# Autodesk Inventor assembly: OUTK_000_Assembly
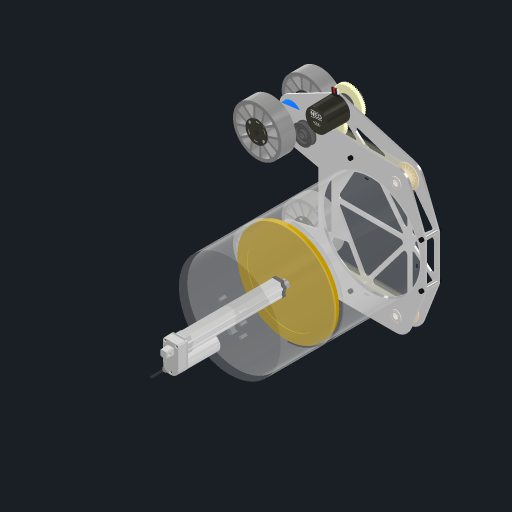
[picture p0: Inventor's stored thumbnail of the model, 512x512]
Saved by Autodesk Inventor 2024.2 (Build 282272000, 272)
## iProperties
Created: 2024-11-24
Part Number: OUTK_000_Assembly
Document SubType Name: Assembly
Designer: Bryan
Mass: 9682.5 g
Surface Area: 20203.5 cm^2
Volume: 5331.75 cm^3
Density: 1.81601 g/cm^3
Author: Bryan
## Documents named in this file (23)
- C:\Users\bobsb\OneDrive\Documents\GitHub\1622-2024-Casino-Clash-CAD-A-Thon\Outtake\OUTK_000_Assembly.iam
- C:\Users\bobsb\OneDrive\Documents\GitHub\1622-2024-Casino-Clash-CAD-A-Thon\Outtake\OUTK_002_ShotPlateNoReceptacle.ipt
- C:\Users\bobsb\OneDrive\Documents\GitHub\1622-2024-Casino-Clash-CAD-A-Thon\Outtake\OUTK_002_ShotPlateReceptacle.ipt
- C:\Users\bobsb\OneDrive\Documents\GitHub\1622-2024-Casino-Clash-CAD-A-Thon\Outtake\OUTK_001_ChipBucket.ipt
- C:\Users\bobsb\OneDrive\Documents\GitHub\1622-2024-Casino-Clash-CAD-A-Thon\COTS Library\Motion\Linear Actuators\PA-01\COTS_PA-01.iam
- C:\Users\bobsb\OneDrive\Documents\GitHub\1622-2024-Casino-Clash-CAD-A-Thon\COTS Library\Motion\Linear Actuators\PA-01\Shaft.ipt
- C:\Users\bobsb\OneDrive\Documents\GitHub\1622-2024-Casino-Clash-CAD-A-Thon\COTS Library\Motion\Bearings\COTS_WCP-0783_1.125ODHexBearing.ipt
- C:\Users\bobsb\OneDrive\Documents\GitHub\1622-2024-Casino-Clash-CAD-A-Thon\COTS Library\Motion\Wheels\Compliant Wheels\5in compliant wheels\COTS_5 Straight Flex Wheel (.ipt
- C:\Users\bobsb\OneDrive\Documents\GitHub\1622-2024-Casino-Clash-CAD-A-Thon\COTS Library\Adapters\COTS_1_2” Hex Bore Aluminum VersaHub (217-2592)(1).ipt
- C:\Users\bobsb\OneDrive\Documents\GitHub\1622-2024-Casino-Clash-CAD-A-Thon\COTS Library\Motion\Wheels\Compliant Wheels\2in compliant wheels\0.500in hex bore\COTS_am-3462_2indiameter_0.500inhexbore_durometer50A_CompliantWheel.ipt
- C:\Users\bobsb\OneDrive\Documents\GitHub\1622-2024-Casino-Clash-CAD-A-Thon\Game Objects\Chip, Simplified.ipt
- C:\Users\bobsb\OneDrive\Documents\GitHub\1622-2024-Casino-Clash-CAD-A-Thon\Outtake\OUTK_010_Grippy.ipt
- C:\Users\bobsb\OneDrive\Documents\GitHub\1622-2024-Casino-Clash-CAD-A-Thon\Outtake\OUTK_011_Tubing.ipt
- C:\Users\bobsb\OneDrive\Documents\GitHub\1622-2024-Casino-Clash-CAD-A-Thon\COTS Library\Fasteners\Bolts\Set Screws\10-32\COTS_91375A446_Alloy Steel Cup-Point Set Screw.ipt
- C:\Users\bobsb\OneDrive\Documents\GitHub\1622-2024-Casino-Clash-CAD-A-Thon\COTS Library\Motion\Pulleys\HTD5M\10mm Wide\COTS_30T_WCP-0565.ipt
- C:\Users\bobsb\OneDrive\Documents\GitHub\1622-2024-Casino-Clash-CAD-A-Thon\COTS Library\Motors\COTS_REV-21-1650-V1.1_Neo1.1.ipt
- C:\Users\bobsb\OneDrive\Documents\GitHub\1622-2024-Casino-Clash-CAD-A-Thon\COTS Library\Fasteners\Bolts\Button-Head\10-32\COTS_91255A265_Button Head Hex Drive Screw.ipt
- C:\Users\bobsb\OneDrive\Documents\GitHub\1622-2024-Casino-Clash-CAD-A-Thon\COTS Library\Adapters\COTS_REV-21-1879_8mmKeyTo0.5Hex.ipt
- C:\Users\bobsb\OneDrive\Documents\GitHub\1622-2024-Casino-Clash-CAD-A-Thon\COTS Library\Motion\Pulleys\HTD5M\10mm Wide\COTS_24T_WCP-0564.ipt
- C:\Users\bobsb\OneDrive\Documents\GitHub\1622-2024-Casino-Clash-CAD-A-Thon\COTS Library\Motion\Gears\20DP gears\Aluminum\0.5in hex\COTS_60T_WCP-0720(1).ipt
- C:\Users\bobsb\OneDrive\Documents\GitHub\1622-2024-Casino-Clash-CAD-A-Thon\Outtake\OUTK_012_Spacer1.ipt
- C:\Users\bobsb\OneDrive\Documents\GitHub\1622-2024-Casino-Clash-CAD-A-Thon\Outtake\OUTK_013_Standoff1.ipt
- C:\Users\bobsb\OneDrive\Documents\GitHub\1622-2024-Casino-Clash-CAD-A-Thon\COTS Library\Fasteners\Bolts\Socket-Head\0.25-20\COTS_91251A537_Black-Oxide Alloy Steel Socket Head Screw_.25-20_.5in.ipt
## Components (116 placed, 22 different names)
1. OUTK_002_ShotPlateNoReceptacle:1 — Mate:4, Mate:5, Mate:41, Mate:47, Mate:50, Mate:52, Mate:55, Mate:56, Mate:57, Mate:65, Mate:66, Mate:67, Mate:68, Mate:69, Mate:70, Mate:149, Mate:150, Mate:151, Mate:152, Mate:153, Mate:169, Mate:170, Mate:171, Mate:172, Mate:173, Mate:174, Mate:175, Mate:176, Mate:177, Mate:178, Mate:181, Mate:182, Mate:187, Mate:188, Mate:189, Mate:192
2. OUTK_002_ShotPlateReceptacle:1 — Mate:3, Mate:4, Mate:5, Mate:41, Mate:42, Mate:48, Mate:49, Mate:51, Mate:53, Mate:54, Mate:58, Mate:59, Mate:60, Mate:61, Mate:62, Mate:63, Mate:64, Mate:141, Mate:179, Mate:180, Mate:183, Mate:184, Mate:185, Mate:186, Mate:190, Mate:191
3. OUTK_001_ChipBucket:1 — Mate:3, Mate:42, Mate:43, Mate:44, Mate:114, Flush:1, Mate:161, Mate:162
4. COTS_PA-01:1 [sub-assembly] — Mate:43, Mate:44, Mate:46, Flush:1
5. Shaft:1 — Mate:46, Mate:115
6. COTS_WCP-0783_1.125ODHexBearing:1 — Mate:47, Mate:65, Mate:72, Mate:107, Mate:166, Mate:168
7. COTS_WCP-0783_1.125ODHexBearing:2 — Mate:48, Mate:62, Mate:74, Mate:106, Mate:108, Mate:145
8. COTS_WCP-0783_1.125ODHexBearing:3 — Mate:49, Mate:64, Mate:120, Mate:143, Mate:146
9. COTS_WCP-0783_1.125ODHexBearing:4 — Mate:50, Mate:66, Mate:124, Mate:156, Mate:157
10. COTS_WCP-0783_1.125ODHexBearing:5 — Mate:51, Mate:63, Mate:117
11. COTS_WCP-0783_1.125ODHexBearing:6 — Mate:52, Mate:67, Mate:123
12. COTS_WCP-0783_1.125ODHexBearing:7 — Mate:55, Mate:69, Mate:122, Mate:160
13. COTS_WCP-0783_1.125ODHexBearing:8 — Mate:56, Mate:68, Mate:71, Mate:110, Mate:111, Mate:163, Mate:165
14. COTS_WCP-0783_1.125ODHexBearing:9 — Mate:53, Mate:61, Mate:119, Mate:142, Mate:144
15. COTS_WCP-0783_1.125ODHexBearing:10 — Mate:54, Mate:60, Mate:73, Mate:112, Mate:139, Mate:140
16. COTS_WCP-0783_1.125ODHexBearing:11 — Mate:57, Mate:70, Mate:121
17. COTS_WCP-0783_1.125ODHexBearing:12 — Mate:58, Mate:59, Mate:118
18. COTS_5 Straight Flex Wheel (:1 — Mate:71, Mate:75, Mate:80, Mate:85, Mate:88, Mate:89, Mate:90
19. COTS_5 Straight Flex Wheel (:2 — Mate:72, Mate:76, Mate:81, Mate:86, Mate:87, Mate:94, Mate:95, Mate:96
20. COTS_5 Straight Flex Wheel (:3 — Mate:73, Mate:78, Mate:79, Mate:84, Mate:91, Mate:92, Mate:93
21. COTS_5 Straight Flex Wheel (:4 — Mate:74, Mate:77, Mate:82, Mate:83, Mate:97, Mate:98, Mate:99
22. COTS_1_2” Hex Bore Aluminum VersaHub (217-2592)(1):1 — Mate:77, Mate:82, Mate:83, Mate:135, Flush:8
23. COTS_1_2” Hex Bore Aluminum VersaHub (217-2592)(1):2 — Mate:76, Mate:81, Mate:86, Mate:87, Mate:130, Flush:3
24. COTS_1_2” Hex Bore Aluminum VersaHub (217-2592)(1):3 — Mate:78, Mate:79, Mate:84, Mate:134, Flush:7
25. COTS_1_2” Hex Bore Aluminum VersaHub (217-2592)(1):4 — Mate:75, Mate:80, Mate:85, Mate:131, Flush:4
26. COTS_1_2” Hex Bore Aluminum VersaHub (217-2592)(1):5 — Mate:88, Mate:89, Mate:90, Mate:132, Flush:5, Mate:164
27. COTS_1_2” Hex Bore Aluminum VersaHub (217-2592)(1):6 — Mate:91, Mate:92, Mate:93, Mate:133, Flush:6, Mate:147
28. COTS_1_2” Hex Bore Aluminum VersaHub (217-2592)(1):7 — Mate:94, Mate:95, Mate:96, Mate:129, Flush:2, Mate:167
29. COTS_1_2” Hex Bore Aluminum VersaHub (217-2592)(1):8 — Mate:97, Mate:98, Mate:99, Mate:136, Flush:9, Mate:148
30. COTS_am-3462_2indiameter_0.500inhexbore_durometer50A_CompliantWheel:1 — Mate:106, Mate:107, Mate:109
31. COTS_am-3462_2indiameter_0.500inhexbore_durometer50A_CompliantWheel:2 — Mate:108, Mate:109
32. COTS_am-3462_2indiameter_0.500inhexbore_durometer50A_CompliantWheel:3 — Mate:110, Mate:111, Mate:113
33. COTS_am-3462_2indiameter_0.500inhexbore_durometer50A_CompliantWheel:4 — Mate:112, Mate:113
34. Chip, Simplified:1 — Mate:114, Mate:115
35. OUTK_010_Grippy:1 — Mate:120, Mate:124, Mate:128
36. OUTK_010_Grippy:2 — Mate:119, Mate:122, Mate:126
37. OUTK_010_Grippy:3 — Mate:118, Mate:121, Mate:125, Tangent:4
38. OUTK_010_Grippy:4 — Mate:117, Mate:123, Mate:127, Tangent:5
39. OUTK_011_Tubing:1 — Mate:125, Mate:126, Tangent:4
40. OUTK_011_Tubing:2 — Mate:127, Mate:128, Tangent:5
41. COTS_30T_WCP-0565:1 — Mate:139, Mate:140, Mate:147
42. COTS_30T_WCP-0565:2 — Mate:141, Mate:145, Mate:148
43. COTS_30T_WCP-0565:3 — Mate:143, Mate:146
44. COTS_30T_WCP-0565:4 — Mate:142, Mate:144
45. COTS_REV-21-1650-V1.1_Neo1.1:1 — Mate:149, Mate:150, Mate:151, Mate:154, Mate:155, Mate:158
46. COTS_REV-21-1879_8mmKeyTo0.5Hex:1 — Mate:154, Flush:11
47. COTS_24T_WCP-0564:1 — Mate:155, Flush:10, Mate:159
48. COTS_24T_WCP-0564:2 — Mate:156, Mate:157, Flush:10
49. COTS_60T_WCP-0720(1):1 — Mate:158, Mate:159, Flush:11, Flush:12
50. COTS_60T_WCP-0720(1):2 — Mate:160, Flush:12
51. OUTK_012_Spacer1:1 — Mate:166, Mate:167, Mate:168
52. OUTK_012_Spacer1:2 — Mate:163, Mate:164, Mate:165
53. OUTK_013_Standoff1:1 — Mate:172, Mate:173
54. OUTK_013_Standoff1:2 — Mate:171, Mate:174
55. OUTK_013_Standoff1:3 — Mate:170, Mate:175
56. OUTK_013_Standoff1:4 — Mate:169, Mate:176
57. COTS_91251A537_Black-Oxide Alloy Steel Socket Head Screw_.25-20_.5in:1 — Mate:177, Mate:178
58. COTS_91251A537_Black-Oxide Alloy Steel Socket Head Screw_.25-20_.5in:2 — Mate:179, Mate:180
59. COTS_91251A537_Black-Oxide Alloy Steel Socket Head Screw_.25-20_.5in:3 — Mate:181, Mate:182
60. COTS_91251A537_Black-Oxide Alloy Steel Socket Head Screw_.25-20_.5in:4 — Mate:183, Mate:184
61. COTS_91251A537_Black-Oxide Alloy Steel Socket Head Screw_.25-20_.5in:5 — Mate:187, Mate:188
62. COTS_91251A537_Black-Oxide Alloy Steel Socket Head Screw_.25-20_.5in:6 — Mate:185, Mate:186
63. COTS_91251A537_Black-Oxide Alloy Steel Socket Head Screw_.25-20_.5in:7 — Mate:189, Mate:192
64. COTS_91251A537_Black-Oxide Alloy Steel Socket Head Screw_.25-20_.5in:8 — Mate:190, Mate:191
65. COTS_91375A446_Alloy Steel Cup-Point Set Screw:13 — Mate:129, Flush:2
66. COTS_91375A446_Alloy Steel Cup-Point Set Screw:14
67. COTS_91375A446_Alloy Steel Cup-Point Set Screw:15
68. COTS_91375A446_Alloy Steel Cup-Point Set Screw:16
69. COTS_91375A446_Alloy Steel Cup-Point Set Screw:17
70. COTS_91375A446_Alloy Steel Cup-Point Set Screw:18
71. COTS_91375A446_Alloy Steel Cup-Point Set Screw:1 — Mate:130, Flush:3
72. COTS_91375A446_Alloy Steel Cup-Point Set Screw:19
73. COTS_91375A446_Alloy Steel Cup-Point Set Screw:20
74. COTS_91375A446_Alloy Steel Cup-Point Set Screw:21
75. COTS_91375A446_Alloy Steel Cup-Point Set Screw:22
76. COTS_91375A446_Alloy Steel Cup-Point Set Screw:23
77. COTS_91375A446_Alloy Steel Cup-Point Set Screw:6 — Mate:131, Flush:4
78. COTS_91375A446_Alloy Steel Cup-Point Set Screw:24
79. COTS_91375A446_Alloy Steel Cup-Point Set Screw:25
80. COTS_91375A446_Alloy Steel Cup-Point Set Screw:26
81. COTS_91375A446_Alloy Steel Cup-Point Set Screw:27
82. COTS_91375A446_Alloy Steel Cup-Point Set Screw:28
83. COTS_91375A446_Alloy Steel Cup-Point Set Screw:7 — Mate:132, Flush:5
84. COTS_91375A446_Alloy Steel Cup-Point Set Screw:29
85. COTS_91375A446_Alloy Steel Cup-Point Set Screw:30
86. COTS_91375A446_Alloy Steel Cup-Point Set Screw:31
87. COTS_91375A446_Alloy Steel Cup-Point Set Screw:32
88. COTS_91375A446_Alloy Steel Cup-Point Set Screw:33
89. COTS_91375A446_Alloy Steel Cup-Point Set Screw:11 — Mate:134, Flush:7
90. COTS_91375A446_Alloy Steel Cup-Point Set Screw:34
91. COTS_91375A446_Alloy Steel Cup-Point Set Screw:35
92. COTS_91375A446_Alloy Steel Cup-Point Set Screw:36
93. COTS_91375A446_Alloy Steel Cup-Point Set Screw:37
94. COTS_91375A446_Alloy Steel Cup-Point Set Screw:38
95. COTS_91375A446_Alloy Steel Cup-Point Set Screw:12 — Mate:133, Flush:6
96. COTS_91375A446_Alloy Steel Cup-Point Set Screw:39
97. COTS_91375A446_Alloy Steel Cup-Point Set Screw:40
98. COTS_91375A446_Alloy Steel Cup-Point Set Screw:41
99. COTS_91375A446_Alloy Steel Cup-Point Set Screw:42
100. COTS_91375A446_Alloy Steel Cup-Point Set Screw:43
101. COTS_91375A446_Alloy Steel Cup-Point Set Screw:9 — Mate:136, Flush:9
102. COTS_91375A446_Alloy Steel Cup-Point Set Screw:44
103. COTS_91375A446_Alloy Steel Cup-Point Set Screw:45
104. COTS_91375A446_Alloy Steel Cup-Point Set Screw:46
105. COTS_91375A446_Alloy Steel Cup-Point Set Screw:47
106. COTS_91375A446_Alloy Steel Cup-Point Set Screw:48
107. COTS_91375A446_Alloy Steel Cup-Point Set Screw:10 — Mate:135, Flush:8
108. COTS_91375A446_Alloy Steel Cup-Point Set Screw:49
109. COTS_91375A446_Alloy Steel Cup-Point Set Screw:50
110. COTS_91375A446_Alloy Steel Cup-Point Set Screw:51
111. COTS_91375A446_Alloy Steel Cup-Point Set Screw:52
112. COTS_91375A446_Alloy Steel Cup-Point Set Screw:53
113. COTS_91255A265_Button Head Hex Drive Screw:1 — Mate:152, Mate:153
114. COTS_91255A265_Button Head Hex Drive Screw:2
115. COTS_91255A265_Button Head Hex Drive Screw:3
116. COTS_91255A265_Button Head Hex Drive Screw:4
## Component patterns: (6 elements, first: COTS_91375A446_Alloy Steel Cup-Point Set Screw:13), (6 elements, first: COTS_91375A446_Alloy Steel Cup-Point Set Screw:1), (6 elements, first: COTS_91375A446_Alloy Steel Cup-Point Set Screw:6), (6 elements, first: COTS_91375A446_Alloy Steel Cup-Point Set Screw:7), (6 elements, first: COTS_91375A446_Alloy Steel Cup-Point Set Screw:11), (6 elements, first: COTS_91375A446_Alloy Steel Cup-Point Set Screw:12), (6 elements, first: COTS_91375A446_Alloy Steel Cup-Point Set Screw:9), (6 elements, first: COTS_91375A446_Alloy Steel Cup-Point Set Screw:10), (4 elements, first: COTS_91255A265_Button Head Hex Drive Screw:1)
## Relationships (160: Mate 145, Flush 12, Tangent 2, Angle 1)
- Mate:3: OUTK_002_ShotPlateReceptacle:1 ↔ OUTK_001_ChipBucket:1
- Mate:4: OUTK_002_ShotPlateNoReceptacle:1 ↔ OUTK_002_ShotPlateReceptacle:1
- Mate:5: OUTK_002_ShotPlateNoReceptacle:1 ↔ OUTK_002_ShotPlateReceptacle:1
- Mate:41 (30.1625 mm): OUTK_002_ShotPlateNoReceptacle:1 ↔ OUTK_002_ShotPlateReceptacle:1
- Mate:42: OUTK_002_ShotPlateReceptacle:1 ↔ OUTK_001_ChipBucket:1
- Mate:43: OUTK_001_ChipBucket:1 ↔ COTS_PA-01:1
- Mate:44: OUTK_001_ChipBucket:1 ↔ COTS_PA-01:1
- Mate:46: COTS_PA-01:1 ↔ Shaft:1
- Mate:47: OUTK_002_ShotPlateNoReceptacle:1 ↔ COTS_WCP-0783_1.125ODHexBearing:1
- Mate:48: OUTK_002_ShotPlateReceptacle:1 ↔ COTS_WCP-0783_1.125ODHexBearing:2
- Mate:49: OUTK_002_ShotPlateReceptacle:1 ↔ COTS_WCP-0783_1.125ODHexBearing:3
- Mate:50: OUTK_002_ShotPlateNoReceptacle:1 ↔ COTS_WCP-0783_1.125ODHexBearing:4
- Mate:51: OUTK_002_ShotPlateReceptacle:1 ↔ COTS_WCP-0783_1.125ODHexBearing:5
- Mate:52: OUTK_002_ShotPlateNoReceptacle:1 ↔ COTS_WCP-0783_1.125ODHexBearing:6
- Mate:53: OUTK_002_ShotPlateReceptacle:1 ↔ COTS_WCP-0783_1.125ODHexBearing:9
- Mate:54: OUTK_002_ShotPlateReceptacle:1 ↔ COTS_WCP-0783_1.125ODHexBearing:10
- Mate:55: OUTK_002_ShotPlateNoReceptacle:1 ↔ COTS_WCP-0783_1.125ODHexBearing:7
- Mate:56: OUTK_002_ShotPlateNoReceptacle:1 ↔ COTS_WCP-0783_1.125ODHexBearing:8
- Mate:57: OUTK_002_ShotPlateNoReceptacle:1 ↔ COTS_WCP-0783_1.125ODHexBearing:11
- Mate:58: OUTK_002_ShotPlateReceptacle:1 ↔ COTS_WCP-0783_1.125ODHexBearing:12
- Mate:59: OUTK_002_ShotPlateReceptacle:1 ↔ COTS_WCP-0783_1.125ODHexBearing:12
- Mate:60: OUTK_002_ShotPlateReceptacle:1 ↔ COTS_WCP-0783_1.125ODHexBearing:10
- Mate:61: OUTK_002_ShotPlateReceptacle:1 ↔ COTS_WCP-0783_1.125ODHexBearing:9
- Mate:62: OUTK_002_ShotPlateReceptacle:1 ↔ COTS_WCP-0783_1.125ODHexBearing:2
- Mate:63: OUTK_002_ShotPlateReceptacle:1 ↔ COTS_WCP-0783_1.125ODHexBearing:5
- Mate:64: OUTK_002_ShotPlateReceptacle:1 ↔ COTS_WCP-0783_1.125ODHexBearing:3
- Mate:65: OUTK_002_ShotPlateNoReceptacle:1 ↔ COTS_WCP-0783_1.125ODHexBearing:1
- Mate:66: OUTK_002_ShotPlateNoReceptacle:1 ↔ COTS_WCP-0783_1.125ODHexBearing:4
- Mate:67: OUTK_002_ShotPlateNoReceptacle:1 ↔ COTS_WCP-0783_1.125ODHexBearing:6
- Mate:68: OUTK_002_ShotPlateNoReceptacle:1 ↔ COTS_WCP-0783_1.125ODHexBearing:8
- Mate:69: OUTK_002_ShotPlateNoReceptacle:1 ↔ COTS_WCP-0783_1.125ODHexBearing:7
- Mate:70: OUTK_002_ShotPlateNoReceptacle:1 ↔ COTS_WCP-0783_1.125ODHexBearing:11
- Mate:71: COTS_WCP-0783_1.125ODHexBearing:8 ↔ COTS_5 Straight Flex Wheel (:1
- Mate:72: COTS_WCP-0783_1.125ODHexBearing:1 ↔ COTS_5 Straight Flex Wheel (:2
- Mate:73: COTS_WCP-0783_1.125ODHexBearing:10 ↔ COTS_5 Straight Flex Wheel (:3
- Mate:74: COTS_WCP-0783_1.125ODHexBearing:2 ↔ COTS_5 Straight Flex Wheel (:4
- Mate:75: COTS_5 Straight Flex Wheel (:1 ↔ COTS_1_2” Hex Bore Aluminum VersaHub (217-2592)(1):4
- Mate:76: COTS_5 Straight Flex Wheel (:2 ↔ COTS_1_2” Hex Bore Aluminum VersaHub (217-2592)(1):2
- Mate:77: COTS_5 Straight Flex Wheel (:4 ↔ COTS_1_2” Hex Bore Aluminum VersaHub (217-2592)(1):1
- Mate:78: COTS_5 Straight Flex Wheel (:3 ↔ COTS_1_2” Hex Bore Aluminum VersaHub (217-2592)(1):3
- Mate:79: COTS_5 Straight Flex Wheel (:3 ↔ COTS_1_2” Hex Bore Aluminum VersaHub (217-2592)(1):3
- Mate:80: COTS_5 Straight Flex Wheel (:1 ↔ COTS_1_2” Hex Bore Aluminum VersaHub (217-2592)(1):4
- Mate:81: COTS_5 Straight Flex Wheel (:2 ↔ COTS_1_2” Hex Bore Aluminum VersaHub (217-2592)(1):2
- Mate:82: COTS_5 Straight Flex Wheel (:4 ↔ COTS_1_2” Hex Bore Aluminum VersaHub (217-2592)(1):1
- Mate:83: COTS_5 Straight Flex Wheel (:4 ↔ COTS_1_2” Hex Bore Aluminum VersaHub (217-2592)(1):1
- Mate:84: COTS_5 Straight Flex Wheel (:3 ↔ COTS_1_2” Hex Bore Aluminum VersaHub (217-2592)(1):3
- Mate:85: COTS_5 Straight Flex Wheel (:1 ↔ COTS_1_2” Hex Bore Aluminum VersaHub (217-2592)(1):4
- Mate:86: COTS_5 Straight Flex Wheel (:2 ↔ COTS_1_2” Hex Bore Aluminum VersaHub (217-2592)(1):2
- Mate:87: COTS_5 Straight Flex Wheel (:2 ↔ COTS_1_2” Hex Bore Aluminum VersaHub (217-2592)(1):2
- Mate:88: COTS_5 Straight Flex Wheel (:1 ↔ COTS_1_2” Hex Bore Aluminum VersaHub (217-2592)(1):5
- Mate:89: COTS_5 Straight Flex Wheel (:1 ↔ COTS_1_2” Hex Bore Aluminum VersaHub (217-2592)(1):5
- Mate:90: COTS_5 Straight Flex Wheel (:1 ↔ COTS_1_2” Hex Bore Aluminum VersaHub (217-2592)(1):5
- Mate:91: COTS_5 Straight Flex Wheel (:3 ↔ COTS_1_2” Hex Bore Aluminum VersaHub (217-2592)(1):6
- Mate:92: COTS_5 Straight Flex Wheel (:3 ↔ COTS_1_2” Hex Bore Aluminum VersaHub (217-2592)(1):6
- Mate:93: COTS_5 Straight Flex Wheel (:3 ↔ COTS_1_2” Hex Bore Aluminum VersaHub (217-2592)(1):6
- Mate:94: COTS_5 Straight Flex Wheel (:2 ↔ COTS_1_2” Hex Bore Aluminum VersaHub (217-2592)(1):7
- Mate:95: COTS_5 Straight Flex Wheel (:2 ↔ COTS_1_2” Hex Bore Aluminum VersaHub (217-2592)(1):7
- Mate:96: COTS_5 Straight Flex Wheel (:2 ↔ COTS_1_2” Hex Bore Aluminum VersaHub (217-2592)(1):7
- Mate:97: COTS_5 Straight Flex Wheel (:4 ↔ COTS_1_2” Hex Bore Aluminum VersaHub (217-2592)(1):8
- Mate:98: COTS_5 Straight Flex Wheel (:4 ↔ COTS_1_2” Hex Bore Aluminum VersaHub (217-2592)(1):8
- Mate:99: COTS_5 Straight Flex Wheel (:4 ↔ COTS_1_2” Hex Bore Aluminum VersaHub (217-2592)(1):8
- Mate:106: COTS_WCP-0783_1.125ODHexBearing:2 ↔ COTS_am-3462_2indiameter_0.500inhexbore_durometer50A_CompliantWheel:1
- Mate:107 (0.7937 mm): COTS_WCP-0783_1.125ODHexBearing:1 ↔ COTS_am-3462_2indiameter_0.500inhexbore_durometer50A_CompliantWheel:1
- Mate:108: COTS_WCP-0783_1.125ODHexBearing:2 ↔ COTS_am-3462_2indiameter_0.500inhexbore_durometer50A_CompliantWheel:2
- Mate:109: COTS_am-3462_2indiameter_0.500inhexbore_durometer50A_CompliantWheel:1 ↔ COTS_am-3462_2indiameter_0.500inhexbore_durometer50A_CompliantWheel:2
- Mate:110: COTS_WCP-0783_1.125ODHexBearing:8 ↔ COTS_am-3462_2indiameter_0.500inhexbore_durometer50A_CompliantWheel:3
- Mate:111 (0.7937 mm): COTS_WCP-0783_1.125ODHexBearing:8 ↔ COTS_am-3462_2indiameter_0.500inhexbore_durometer50A_CompliantWheel:3
- Mate:112: COTS_WCP-0783_1.125ODHexBearing:10 ↔ COTS_am-3462_2indiameter_0.500inhexbore_durometer50A_CompliantWheel:4
- Mate:113: COTS_am-3462_2indiameter_0.500inhexbore_durometer50A_CompliantWheel:3 ↔ COTS_am-3462_2indiameter_0.500inhexbore_durometer50A_CompliantWheel:4
- Mate:114: OUTK_001_ChipBucket:1 ↔ Chip, Simplified:1
- Mate:115: Shaft:1 ↔ Chip, Simplified:1
- Flush:1 (15.875 mm): OUTK_001_ChipBucket:1 ↔ COTS_PA-01:1
- Mate:117: COTS_WCP-0783_1.125ODHexBearing:5 ↔ OUTK_010_Grippy:4
- Mate:118: COTS_WCP-0783_1.125ODHexBearing:12 ↔ OUTK_010_Grippy:3
- Mate:119: COTS_WCP-0783_1.125ODHexBearing:9 ↔ OUTK_010_Grippy:2
- Mate:120: COTS_WCP-0783_1.125ODHexBearing:3 ↔ OUTK_010_Grippy:1
- Mate:121 (0.7937 mm): COTS_WCP-0783_1.125ODHexBearing:11 ↔ OUTK_010_Grippy:3
- Mate:122 (0.7937 mm): COTS_WCP-0783_1.125ODHexBearing:7 ↔ OUTK_010_Grippy:2
- Mate:123 (0.7937 mm): COTS_WCP-0783_1.125ODHexBearing:6 ↔ OUTK_010_Grippy:4
- Mate:124 (0.7937 mm): COTS_WCP-0783_1.125ODHexBearing:4 ↔ OUTK_010_Grippy:1
- Mate:125: OUTK_010_Grippy:3 ↔ OUTK_011_Tubing:1
- Mate:126: OUTK_010_Grippy:2 ↔ OUTK_011_Tubing:1
- Tangent:4: OUTK_010_Grippy:3 ↔ OUTK_011_Tubing:1
- Mate:127: OUTK_010_Grippy:4 ↔ OUTK_011_Tubing:2
- Mate:128: OUTK_010_Grippy:1 ↔ OUTK_011_Tubing:2
- Tangent:5: OUTK_010_Grippy:4 ↔ OUTK_011_Tubing:2
- Mate:129: COTS_1_2” Hex Bore Aluminum VersaHub (217-2592)(1):7 ↔ COTS_91375A446_Alloy Steel Cup-Point Set Screw:13
- Flush:2: COTS_1_2” Hex Bore Aluminum VersaHub (217-2592)(1):7 ↔ COTS_91375A446_Alloy Steel Cup-Point Set Screw:13
- Mate:130: COTS_1_2” Hex Bore Aluminum VersaHub (217-2592)(1):2 ↔ COTS_91375A446_Alloy Steel Cup-Point Set Screw:1
- Flush:3: COTS_1_2” Hex Bore Aluminum VersaHub (217-2592)(1):2 ↔ COTS_91375A446_Alloy Steel Cup-Point Set Screw:1
- Mate:131: COTS_1_2” Hex Bore Aluminum VersaHub (217-2592)(1):4 ↔ COTS_91375A446_Alloy Steel Cup-Point Set Screw:6
- Flush:4: COTS_1_2” Hex Bore Aluminum VersaHub (217-2592)(1):4 ↔ COTS_91375A446_Alloy Steel Cup-Point Set Screw:6
- Mate:132: COTS_1_2” Hex Bore Aluminum VersaHub (217-2592)(1):5 ↔ COTS_91375A446_Alloy Steel Cup-Point Set Screw:7
- Flush:5: COTS_1_2” Hex Bore Aluminum VersaHub (217-2592)(1):5 ↔ COTS_91375A446_Alloy Steel Cup-Point Set Screw:7
- Mate:133: COTS_1_2” Hex Bore Aluminum VersaHub (217-2592)(1):6 ↔ COTS_91375A446_Alloy Steel Cup-Point Set Screw:12
- Flush:6: COTS_1_2” Hex Bore Aluminum VersaHub (217-2592)(1):6 ↔ COTS_91375A446_Alloy Steel Cup-Point Set Screw:12
- Mate:134: COTS_1_2” Hex Bore Aluminum VersaHub (217-2592)(1):3 ↔ COTS_91375A446_Alloy Steel Cup-Point Set Screw:11
- Flush:7: COTS_1_2” Hex Bore Aluminum VersaHub (217-2592)(1):3 ↔ COTS_91375A446_Alloy Steel Cup-Point Set Screw:11
- Mate:135: COTS_1_2” Hex Bore Aluminum VersaHub (217-2592)(1):1 ↔ COTS_91375A446_Alloy Steel Cup-Point Set Screw:10
- Flush:8: COTS_1_2” Hex Bore Aluminum VersaHub (217-2592)(1):1 ↔ COTS_91375A446_Alloy Steel Cup-Point Set Screw:10
- Mate:136: COTS_1_2” Hex Bore Aluminum VersaHub (217-2592)(1):8 ↔ COTS_91375A446_Alloy Steel Cup-Point Set Screw:9
- Flush:9: COTS_1_2” Hex Bore Aluminum VersaHub (217-2592)(1):8 ↔ COTS_91375A446_Alloy Steel Cup-Point Set Screw:9
- Mate:139: COTS_WCP-0783_1.125ODHexBearing:10 ↔ COTS_30T_WCP-0565:1
- Mate:140: COTS_WCP-0783_1.125ODHexBearing:10 ↔ COTS_30T_WCP-0565:1
- Mate:141: OUTK_002_ShotPlateReceptacle:1 ↔ COTS_30T_WCP-0565:2
- Mate:142: COTS_WCP-0783_1.125ODHexBearing:9 ↔ COTS_30T_WCP-0565:4
- Mate:143: COTS_WCP-0783_1.125ODHexBearing:3 ↔ COTS_30T_WCP-0565:3
- Mate:144: COTS_WCP-0783_1.125ODHexBearing:9 ↔ COTS_30T_WCP-0565:4
- Mate:145: COTS_WCP-0783_1.125ODHexBearing:2 ↔ COTS_30T_WCP-0565:2
- Mate:146: COTS_WCP-0783_1.125ODHexBearing:3 ↔ COTS_30T_WCP-0565:3
- Mate:147: COTS_1_2” Hex Bore Aluminum VersaHub (217-2592)(1):6 ↔ COTS_30T_WCP-0565:1
- Mate:148: COTS_1_2” Hex Bore Aluminum VersaHub (217-2592)(1):8 ↔ COTS_30T_WCP-0565:2
- Mate:149: OUTK_002_ShotPlateNoReceptacle:1 ↔ COTS_REV-21-1650-V1.1_Neo1.1:1
- Mate:150: OUTK_002_ShotPlateNoReceptacle:1 ↔ COTS_REV-21-1650-V1.1_Neo1.1:1
- Mate:151: OUTK_002_ShotPlateNoReceptacle:1 ↔ COTS_REV-21-1650-V1.1_Neo1.1:1
- Mate:152: OUTK_002_ShotPlateNoReceptacle:1 ↔ COTS_91255A265_Button Head Hex Drive Screw:1
- Mate:153: OUTK_002_ShotPlateNoReceptacle:1 ↔ COTS_91255A265_Button Head Hex Drive Screw:1
- Mate:154: COTS_REV-21-1650-V1.1_Neo1.1:1 ↔ COTS_REV-21-1879_8mmKeyTo0.5Hex:1
- Mate:155: COTS_REV-21-1650-V1.1_Neo1.1:1 ↔ COTS_24T_WCP-0564:1
- Mate:156: COTS_WCP-0783_1.125ODHexBearing:4 ↔ COTS_24T_WCP-0564:2
- Mate:157: COTS_WCP-0783_1.125ODHexBearing:4 ↔ COTS_24T_WCP-0564:2
- Flush:10: COTS_24T_WCP-0564:1 ↔ COTS_24T_WCP-0564:2
- Mate:158: COTS_REV-21-1650-V1.1_Neo1.1:1 ↔ COTS_60T_WCP-0720(1):1
- Mate:159: COTS_24T_WCP-0564:1 ↔ COTS_60T_WCP-0720(1):1
- Flush:11: COTS_REV-21-1879_8mmKeyTo0.5Hex:1 ↔ COTS_60T_WCP-0720(1):1
- Mate:160: COTS_WCP-0783_1.125ODHexBearing:7 ↔ COTS_60T_WCP-0720(1):2
- Flush:12: COTS_60T_WCP-0720(1):1 ↔ COTS_60T_WCP-0720(1):2
- Mate:161: OUTK_001_ChipBucket:1
- Angle:1 (0 deg)
- Mate:162: OUTK_001_ChipBucket:1
- Mate:163: COTS_WCP-0783_1.125ODHexBearing:8 ↔ OUTK_012_Spacer1:2
- Mate:164: COTS_1_2” Hex Bore Aluminum VersaHub (217-2592)(1):5 ↔ OUTK_012_Spacer1:2
- Mate:165: COTS_WCP-0783_1.125ODHexBearing:8 ↔ OUTK_012_Spacer1:2
- Mate:166: COTS_WCP-0783_1.125ODHexBearing:1 ↔ OUTK_012_Spacer1:1
- Mate:167: COTS_1_2” Hex Bore Aluminum VersaHub (217-2592)(1):7 ↔ OUTK_012_Spacer1:1
- Mate:168: COTS_WCP-0783_1.125ODHexBearing:1 ↔ OUTK_012_Spacer1:1
- Mate:169: OUTK_002_ShotPlateNoReceptacle:1 ↔ OUTK_013_Standoff1:4
- Mate:170: OUTK_002_ShotPlateNoReceptacle:1 ↔ OUTK_013_Standoff1:3
- Mate:171: OUTK_002_ShotPlateNoReceptacle:1 ↔ OUTK_013_Standoff1:2
- Mate:172: OUTK_002_ShotPlateNoReceptacle:1 ↔ OUTK_013_Standoff1:1
- Mate:173: OUTK_002_ShotPlateNoReceptacle:1 ↔ OUTK_013_Standoff1:1
- Mate:174: OUTK_002_ShotPlateNoReceptacle:1 ↔ OUTK_013_Standoff1:2
- Mate:175: OUTK_002_ShotPlateNoReceptacle:1 ↔ OUTK_013_Standoff1:3
- Mate:176: OUTK_002_ShotPlateNoReceptacle:1 ↔ OUTK_013_Standoff1:4
- Mate:177: OUTK_002_ShotPlateNoReceptacle:1 ↔ COTS_91251A537_Black-Oxide Alloy Steel Socket Head Screw_.25-20_.5in:1
- Mate:178: OUTK_002_ShotPlateNoReceptacle:1 ↔ COTS_91251A537_Black-Oxide Alloy Steel Socket Head Screw_.25-20_.5in:1
- Mate:179: OUTK_002_ShotPlateReceptacle:1 ↔ COTS_91251A537_Black-Oxide Alloy Steel Socket Head Screw_.25-20_.5in:2
- Mate:180: OUTK_002_ShotPlateReceptacle:1 ↔ COTS_91251A537_Black-Oxide Alloy Steel Socket Head Screw_.25-20_.5in:2
- Mate:181: OUTK_002_ShotPlateNoReceptacle:1 ↔ COTS_91251A537_Black-Oxide Alloy Steel Socket Head Screw_.25-20_.5in:3
- Mate:182: OUTK_002_ShotPlateNoReceptacle:1 ↔ COTS_91251A537_Black-Oxide Alloy Steel Socket Head Screw_.25-20_.5in:3
- Mate:183: OUTK_002_ShotPlateReceptacle:1 ↔ COTS_91251A537_Black-Oxide Alloy Steel Socket Head Screw_.25-20_.5in:4
- Mate:184: OUTK_002_ShotPlateReceptacle:1 ↔ COTS_91251A537_Black-Oxide Alloy Steel Socket Head Screw_.25-20_.5in:4
- Mate:185: OUTK_002_ShotPlateReceptacle:1 ↔ COTS_91251A537_Black-Oxide Alloy Steel Socket Head Screw_.25-20_.5in:6
- Mate:186: OUTK_002_ShotPlateReceptacle:1 ↔ COTS_91251A537_Black-Oxide Alloy Steel Socket Head Screw_.25-20_.5in:6
- Mate:187: OUTK_002_ShotPlateNoReceptacle:1 ↔ COTS_91251A537_Black-Oxide Alloy Steel Socket Head Screw_.25-20_.5in:5
- Mate:188: OUTK_002_ShotPlateNoReceptacle:1 ↔ COTS_91251A537_Black-Oxide Alloy Steel Socket Head Screw_.25-20_.5in:5
- Mate:189: OUTK_002_ShotPlateNoReceptacle:1 ↔ COTS_91251A537_Black-Oxide Alloy Steel Socket Head Screw_.25-20_.5in:7
- Mate:190: OUTK_002_ShotPlateReceptacle:1 ↔ COTS_91251A537_Black-Oxide Alloy Steel Socket Head Screw_.25-20_.5in:8
- Mate:191: OUTK_002_ShotPlateReceptacle:1 ↔ COTS_91251A537_Black-Oxide Alloy Steel Socket Head Screw_.25-20_.5in:8
- Mate:192: OUTK_002_ShotPlateNoReceptacle:1 ↔ COTS_91251A537_Black-Oxide Alloy Steel Socket Head Screw_.25-20_.5in:7
